# Autodesk Inventor assembly: GFRP_T2_04
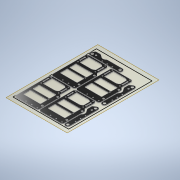
[picture p0: Inventor's stored thumbnail of the model, 180x180]
Saved by Autodesk Inventor 2022.3 (Build 263350000, 350)
## iProperties
Created: 2022-09-28
Part Number: GFRP_T2_04
Document SubType Name: Assembly
Designer: Masato
Author: Masato
## Documents named in this file (4)
- C:\Users\Masato\Documents\Inventor\Inventor for CIT Brains\SUSTAINA-OP - cam\Cam\GFRP_T2\OriginalMind_RD400\GFRP_T2_04.iam
- C:\Users\Masato\Documents\Inventor\Inventor for CIT Brains\SUSTAINA-OP - cam\Cam\DisposableBoard.ipt
- C:\Users\Masato\Documents\Inventor\Inventor for CIT Brains\SUSTAINA-OP - cam\LowerBody\Link\BackLink_frame.ipt
- C:\Users\Masato\Documents\Inventor\Inventor for CIT Brains\SUSTAINA-OP - cam\UpperBody\Trunk\Trunk_upper_side_frame.ipt
## Components (8 placed, 3 different names)
1. DisposableBoard:1 — フラッシュ:1, フラッシュ:2, フラッシュ:3, フラッシュ:4, フラッシュ:12, フラッシュ:13
2. BackLink_frame:2 — メイト:30, メイト:31, 正接:2
3. Trunk_upper_side_frame:1 — メイト:27, フラッシュ:12, フラッシュ:13
4. Trunk_upper_side_frame:2 — メイト:29, 正接:1
5. Trunk_upper_side_frame:3 — メイト:31, 正接:2
6. Trunk_upper_side_frame:4
7. BackLink_frame:1 — メイト:28, メイト:29, 正接:1
8. BackLink_frame:6
## Component patterns: コンポーネント パターン 1:1 (4 elements), コンポーネント パターン 2:1 (2 elements)
## Relationships (13: Flush 6, Mate 5, Tangent 2)
- フラッシュ:1 [Flush]: DisposableBoard:1
- フラッシュ:2 [Flush]: DisposableBoard:1
- フラッシュ:3 [Flush]: DisposableBoard:1
- フラッシュ:4 [Flush]: DisposableBoard:1
- メイト:27 [Mate]: Trunk_upper_side_frame:1
- フラッシュ:12 [Flush] (-2 mm): DisposableBoard:1 ↔ Trunk_upper_side_frame:1
- フラッシュ:13 [Flush] (-2 mm): DisposableBoard:1 ↔ Trunk_upper_side_frame:1
- メイト:28 [Mate]: BackLink_frame:1
- メイト:29 [Mate] (2.1 mm): Trunk_upper_side_frame:2 ↔ BackLink_frame:1
- 正接:1 [Tangent]: Trunk_upper_side_frame:2 ↔ BackLink_frame:1
- メイト:30 [Mate]: BackLink_frame:2
- メイト:31 [Mate] (2.1 mm): BackLink_frame:2 ↔ Trunk_upper_side_frame:3
- 正接:2 [Tangent]: BackLink_frame:2 ↔ Trunk_upper_side_frame:3
